# Autodesk Inventor assembly: bepf_podwozie
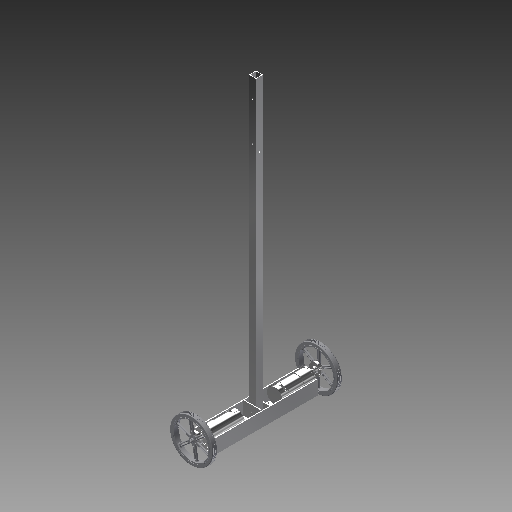
[picture p0: Inventor's stored thumbnail of the model, 512x512]
Saved by Autodesk Inventor 2017 (Build 210142000, 142)
## iProperties
Part Number: bepf_podwozie
Material: Ogólny
Document SubType Name: Assembly
Designer: gagato
Author: gagato
## Documents named in this file (7)
- C:\Users\gagato\Documents\bepf\bepf_podwozie.iam
- C:\Users\gagato\Documents\bepf\bepf_glowny_wspornik.ipt
- C:\Users\gagato\Documents\bepf\bepf_podwozie_lacznik_glownego_wspornika.ipt
- C:\Users\gagato\Documents\bepf\bepf_podwozie_belka_glowna.ipt
- C:\Users\gagato\Documents\bepf\bepf_podwozie_lacznik_silnika.ipt
- C:\Users\gagato\Documents\bepf\bepf_silnik_dc.ipt
- C:\Users\gagato\Documents\bepf\bepf_kolo.iam
## Components (11 placed, 6 different names)
1. bepf_glowny_wspornik:1 — Zestawiający:1, Zestawiający:2, Zestawiający:3, Zestawiający:4, Zestawiający:5, Równoległy:1, Równoległy:2
2. wspornik_nogi_30L20:1 — Zestawiający:2, Zestawiający:3, Równoległy:2, Zestawiający:7, Zestawiający:8, Zestawiający:10, Zestawiający:11
3. wspornik_nogi_30L20:2 — Zestawiający:4, Zestawiający:5, Równoległy:1, Zestawiający:6, Zestawiający:9
4. bepf_podwozie_belka_glowna:1 — Zestawiający:9, Zestawiający:10, Zestawiający:11, Zestawiający:12, Zestawiający:14
5. bepf_podwozie_belka_glowna:2 — Zestawiający:6, Zestawiający:7, Zestawiający:8, Zestawiający:13, Zestawiający:15, Zestawiający:16, Zestawiający:17
6. bepf_podwozie_lacznik_silnika:1 — Zestawiający:12, Zestawiający:13, Zestawiający:17, Zestawiający:18, Zestawiający:19, Zestawiający:20
7. bepf_podwozie_lacznik_silnika:2 — Zestawiający:14, Zestawiający:15, Zestawiający:16, Zestawiający:21, Zestawiający:22, Zestawiający:23
8. bepf_silnik_dc:1 — Zestawiający:18, Zestawiający:19, Zestawiający:20, Zestawiający:24, Zestawiający:25
9. bepf_silnik_dc:2 — Zestawiający:21, Zestawiający:22, Zestawiający:23, Zestawiający:26, Zestawiający:27
10. bepf_kolo:1 [sub-assembly] — Zestawiający:24, Zestawiający:25
11. bepf_kolo:2 [sub-assembly] — Zestawiający:26, Zestawiający:27
## Relationships (29: Mate 27, Flush 2)
- Zestawiający:1 [Mate]: bepf_glowny_wspornik:1
- Zestawiający:2 [Mate]: bepf_glowny_wspornik:1 ↔ wspornik_nogi_30L20:1
- Zestawiający:3 [Mate]: bepf_glowny_wspornik:1 ↔ wspornik_nogi_30L20:1
- Zestawiający:4 [Mate]: bepf_glowny_wspornik:1 ↔ wspornik_nogi_30L20:2
- Zestawiający:5 [Mate]: bepf_glowny_wspornik:1 ↔ wspornik_nogi_30L20:2
- Równoległy:1 [Flush]: bepf_glowny_wspornik:1 ↔ wspornik_nogi_30L20:2
- Równoległy:2 [Flush]: bepf_glowny_wspornik:1 ↔ wspornik_nogi_30L20:1
- Zestawiający:6 [Mate]: wspornik_nogi_30L20:2 ↔ bepf_podwozie_belka_glowna:2
- Zestawiający:7 [Mate]: wspornik_nogi_30L20:1 ↔ bepf_podwozie_belka_glowna:2
- Zestawiający:8 [Mate]: wspornik_nogi_30L20:1 ↔ bepf_podwozie_belka_glowna:2
- Zestawiający:9 [Mate]: wspornik_nogi_30L20:2 ↔ bepf_podwozie_belka_glowna:1
- Zestawiający:10 [Mate]: wspornik_nogi_30L20:1 ↔ bepf_podwozie_belka_glowna:1
- Zestawiający:11 [Mate]: wspornik_nogi_30L20:1 ↔ bepf_podwozie_belka_glowna:1
- Zestawiający:12 [Mate]: bepf_podwozie_belka_glowna:1 ↔ bepf_podwozie_lacznik_silnika:1
- Zestawiający:13 [Mate]: bepf_podwozie_belka_glowna:2 ↔ bepf_podwozie_lacznik_silnika:1
- Zestawiający:14 [Mate]: bepf_podwozie_belka_glowna:1 ↔ bepf_podwozie_lacznik_silnika:2
- Zestawiający:15 [Mate]: bepf_podwozie_belka_glowna:2 ↔ bepf_podwozie_lacznik_silnika:2
- Zestawiający:16 [Mate]: bepf_podwozie_belka_glowna:2 ↔ bepf_podwozie_lacznik_silnika:2
- Zestawiający:17 [Mate]: bepf_podwozie_belka_glowna:2 ↔ bepf_podwozie_lacznik_silnika:1
- Zestawiający:18 [Mate]: bepf_podwozie_lacznik_silnika:1 ↔ bepf_silnik_dc:1
- Zestawiający:19 [Mate]: bepf_podwozie_lacznik_silnika:1 ↔ bepf_silnik_dc:1
- Zestawiający:20 [Mate]: bepf_podwozie_lacznik_silnika:1 ↔ bepf_silnik_dc:1
- Zestawiający:21 [Mate]: bepf_podwozie_lacznik_silnika:2 ↔ bepf_silnik_dc:2
- Zestawiający:22 [Mate]: bepf_podwozie_lacznik_silnika:2 ↔ bepf_silnik_dc:2
- Zestawiający:23 [Mate]: bepf_podwozie_lacznik_silnika:2 ↔ bepf_silnik_dc:2
- Zestawiający:24 [Mate]: bepf_silnik_dc:1 ↔ bepf_kolo:1
- Zestawiający:25 [Mate]: bepf_silnik_dc:1 ↔ bepf_kolo:1
- Zestawiający:26 [Mate]: bepf_silnik_dc:2 ↔ bepf_kolo:2
- Zestawiający:27 [Mate]: bepf_silnik_dc:2 ↔ bepf_kolo:2
